# Autodesk Inventor assembly: Assembly3
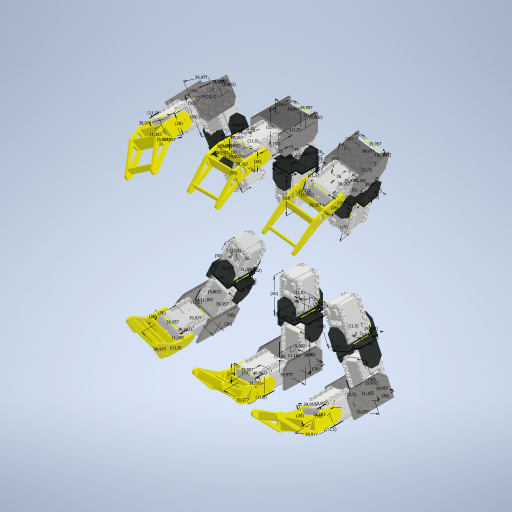
[picture p0: Inventor's stored thumbnail of the model, 512x512]
Saved by Autodesk Inventor 2024 (Build 280153000, 153)
## iProperties
Created: 2024-02-16
Part Number: Assembly3
Document SubType Name: Assembly
Designer: kamil
Author: kamil
## Documents named in this file (5)
- D:\Projects\Robotics\Hexapod\Assembly3.iam
- D:\Projects\Robotics\Hexapod\first_junction.ipt
- D:\Projects\Robotics\Hexapod\AX-12A\AX-12A.iam
- D:\Projects\Robotics\Hexapod\second_junction.ipt
- D:\Projects\Robotics\Hexapod\leg_part.ipt
## Components (36 placed, 4 different names)
1. first_junction:1 — Mate:1, Mate:2, Mate:3, Mate:4, Mate:5, Mate:6, Mate:7
2. AX-12A:1 [sub-assembly] — Mate:1, Mate:2, Mate:3, Mate:4
3. AX-12A:2 [sub-assembly] — Mate:5, Mate:6, Mate:7, Mate:14, Mate:18, Mate:19
4. second_junction:1 — Mate:11, Mate:12, Mate:13, Mate:14, Mate:18, Mate:19
5. AX-12A:3 [sub-assembly] — Mate:11, Mate:12, Mate:13, Mate:15, Mate:16, Mate:17
6. leg_part:1 — Mate:15, Mate:16, Mate:17
7. first_junction:2
8. AX-12A:4 [sub-assembly]
9. AX-12A:5 [sub-assembly]
10. second_junction:2
11. AX-12A:6 [sub-assembly]
12. leg_part:2
13. first_junction:3
14. AX-12A:7 [sub-assembly]
15. AX-12A:8 [sub-assembly]
16. second_junction:3
17. AX-12A:9 [sub-assembly]
18. leg_part:3
19. first_junction:4
20. AX-12A:10 [sub-assembly]
21. AX-12A:11 [sub-assembly]
22. second_junction:4
23. AX-12A:12 [sub-assembly]
24. leg_part:4
25. first_junction:5
26. AX-12A:13 [sub-assembly]
27. AX-12A:14 [sub-assembly]
28. second_junction:5
29. AX-12A:15 [sub-assembly]
30. leg_part:5
31. first_junction:6
32. AX-12A:16 [sub-assembly]
33. AX-12A:17 [sub-assembly]
34. second_junction:6
35. AX-12A:18 [sub-assembly]
36. leg_part:6
## Relationships (96: Mate 96)
- Mate:1: first_junction:1 ↔ AX-12A:1
- Mate:2: first_junction:1 ↔ AX-12A:1
- Mate:3: first_junction:1 ↔ AX-12A:1
- Mate:4: first_junction:1 ↔ AX-12A:1
- Mate:5: first_junction:1 ↔ AX-12A:2
- Mate:6: first_junction:1 ↔ AX-12A:2
- Mate:7: first_junction:1 ↔ AX-12A:2
- Mate:11: second_junction:1 ↔ AX-12A:3
- Mate:12: second_junction:1 ↔ AX-12A:3
- Mate:13: second_junction:1 ↔ AX-12A:3
- Mate:14: AX-12A:2 ↔ second_junction:1
- Mate:15: AX-12A:3 ↔ leg_part:1
- Mate:16: AX-12A:3 ↔ leg_part:1
- Mate:17: AX-12A:3 ↔ leg_part:1
- Mate:18: AX-12A:2 ↔ second_junction:1
- Mate:19: AX-12A:2 ↔ second_junction:1
- [Mate]: first_junction:2 ↔ AX-12A:4
- [Mate]: first_junction:2 ↔ AX-12A:4
- [Mate]: first_junction:2 ↔ AX-12A:4
- [Mate]: first_junction:2 ↔ AX-12A:4
- [Mate]: first_junction:2 ↔ AX-12A:5
- [Mate]: first_junction:2 ↔ AX-12A:5
- [Mate]: first_junction:2 ↔ AX-12A:5
- [Mate]: second_junction:2 ↔ AX-12A:6
- [Mate]: second_junction:2 ↔ AX-12A:6
- [Mate]: second_junction:2 ↔ AX-12A:6
- [Mate]: AX-12A:5 ↔ second_junction:2
- [Mate]: AX-12A:6 ↔ leg_part:2
- [Mate]: AX-12A:6 ↔ leg_part:2
- [Mate]: AX-12A:6 ↔ leg_part:2
- [Mate]: AX-12A:5 ↔ second_junction:2
- [Mate]: AX-12A:5 ↔ second_junction:2
- [Mate]: first_junction:3 ↔ AX-12A:7
- [Mate]: first_junction:3 ↔ AX-12A:7
- [Mate]: first_junction:3 ↔ AX-12A:7
- [Mate]: first_junction:3 ↔ AX-12A:7
- [Mate]: first_junction:3 ↔ AX-12A:8
- [Mate]: first_junction:3 ↔ AX-12A:8
- [Mate]: first_junction:3 ↔ AX-12A:8
- [Mate]: second_junction:3 ↔ AX-12A:9
- [Mate]: second_junction:3 ↔ AX-12A:9
- [Mate]: second_junction:3 ↔ AX-12A:9
- [Mate]: AX-12A:8 ↔ second_junction:3
- [Mate]: AX-12A:9 ↔ leg_part:3
- [Mate]: AX-12A:9 ↔ leg_part:3
- [Mate]: AX-12A:9 ↔ leg_part:3
- [Mate]: AX-12A:8 ↔ second_junction:3
- [Mate]: AX-12A:8 ↔ second_junction:3
- [Mate]: first_junction:4 ↔ AX-12A:10
- [Mate]: first_junction:4 ↔ AX-12A:10
- [Mate]: first_junction:4 ↔ AX-12A:10
- [Mate]: first_junction:4 ↔ AX-12A:10
- [Mate]: first_junction:4 ↔ AX-12A:11
- [Mate]: first_junction:4 ↔ AX-12A:11
- [Mate]: first_junction:4 ↔ AX-12A:11
- [Mate]: second_junction:4 ↔ AX-12A:12
- [Mate]: second_junction:4 ↔ AX-12A:12
- [Mate]: second_junction:4 ↔ AX-12A:12
- [Mate]: AX-12A:11 ↔ second_junction:4
- [Mate]: AX-12A:12 ↔ leg_part:4
- [Mate]: AX-12A:12 ↔ leg_part:4
- [Mate]: AX-12A:12 ↔ leg_part:4
- [Mate]: AX-12A:11 ↔ second_junction:4
- [Mate]: AX-12A:11 ↔ second_junction:4
- [Mate]: first_junction:5 ↔ AX-12A:13
- [Mate]: first_junction:5 ↔ AX-12A:13
- [Mate]: first_junction:5 ↔ AX-12A:13
- [Mate]: first_junction:5 ↔ AX-12A:13
- [Mate]: first_junction:5 ↔ AX-12A:14
- [Mate]: first_junction:5 ↔ AX-12A:14
- [Mate]: first_junction:5 ↔ AX-12A:14
- [Mate]: second_junction:5 ↔ AX-12A:15
- [Mate]: second_junction:5 ↔ AX-12A:15
- [Mate]: second_junction:5 ↔ AX-12A:15
- [Mate]: AX-12A:14 ↔ second_junction:5
- [Mate]: AX-12A:15 ↔ leg_part:5
- [Mate]: AX-12A:15 ↔ leg_part:5
- [Mate]: AX-12A:15 ↔ leg_part:5
- [Mate]: AX-12A:14 ↔ second_junction:5
- [Mate]: AX-12A:14 ↔ second_junction:5
- [Mate]: first_junction:6 ↔ AX-12A:16
- [Mate]: first_junction:6 ↔ AX-12A:16
- [Mate]: first_junction:6 ↔ AX-12A:16
- [Mate]: first_junction:6 ↔ AX-12A:16
- [Mate]: first_junction:6 ↔ AX-12A:17
- [Mate]: first_junction:6 ↔ AX-12A:17
- [Mate]: first_junction:6 ↔ AX-12A:17
- [Mate]: second_junction:6 ↔ AX-12A:18
- [Mate]: second_junction:6 ↔ AX-12A:18
- [Mate]: second_junction:6 ↔ AX-12A:18
- [Mate]: AX-12A:17 ↔ second_junction:6
- [Mate]: AX-12A:18 ↔ leg_part:6
- [Mate]: AX-12A:18 ↔ leg_part:6
- [Mate]: AX-12A:18 ↔ leg_part:6
- [Mate]: AX-12A:17 ↔ second_junction:6
- [Mate]: AX-12A:17 ↔ second_junction:6
## Named parameters: d19_d12 = 0 mm, d20_d13 = 0 mm, d21_d14 = 0 mm, d22_d15 = 0 mm, d23_d16 = 0 mm, d24_d17 = 0 mm, d25_d18 = 0 mm, d26_d0 = 0 mm, d27_d1 = 0 mm, d28_d2 = 0 mm, d29_d3 = 0 mm, d30_d4 = 0 mm, d31_d5 = 0 mm, d32_d6 = 0 mm, d33_d10 = 0 mm, d34_d11 = 0 mm, d35_d12 = 0 mm, d36_d13 = 0 mm, d37_d14 = 0 mm, d38_d15 = 0 mm, d39_d16 = 0 mm, d40_d17 = 0 mm, d41_d18 = 0 mm, d42_d0 = 0 mm, d43_d1 = 0 mm, d44_d2 = 0 mm, d45_d3 = 0 mm, d46_d4 = 0 mm, d47_d5 = 0 mm, d48_d6 = 0 mm, d49_d10 = 0 mm, d50_d11 = 0 mm, d51_d12 = 0 mm, d52_d13 = 0 mm, d53_d14 = 0 mm, d54_d15 = 0 mm, d55_d16 = 0 mm, d56_d17 = 0 mm, d57_d18 = 0 mm, d58_d19_d12 = 0 mm, d59_d20_d13 = 0 mm, d60_d21_d14 = 0 mm, d61_d22_d15 = 0 mm, d62_d23_d16 = 0 mm, d63_d24_d17 = 0 mm, d64_d25_d18 = 0 mm, d65_d26_d0 = 0 mm, d66_d27_d1 = 0 mm, d67_d28_d2 = 0 mm, d68_d29_d3 = 0 mm, d69_d30_d4 = 0 mm, d70_d31_d5 = 0 mm, d71_d32_d6 = 0 mm, d72_d33_d10 = 0 mm, d73_d34_d11 = 0 mm, d74_d35_d12 = 0 mm, d75_d36_d13 = 0 mm, d76_d37_d14 = 0 mm, d77_d0 = 0 mm, d78_d1 = 0 mm, d79_d2 = 0 mm, d80_d3 = 0 mm, d81_d4 = 0 mm, d82_d5 = 0 mm, d83_d6 = 0 mm, d84_d10 = 0 mm, d85_d11 = 0 mm, d86_d38_d15 = 0 mm, d87_d39_d16 = 0 mm, d88_d40_d17 = 0 mm, d89_d41_d18 = 0 mm, d90_d42_d0 = 0 mm, d91_d43_d1 = 0 mm, d92_d44_d2 = 0 mm, d93_d45_d3 = 0 mm, d94_d46_d4 = 0 mm, d95_d47_d5 = 0 mm, d96_d48_d6 = 0 mm, d97_d49_d10 = 0 mm, d98_d50_d11 = 0 mm
